# Autodesk Inventor assembly: feildAssembly
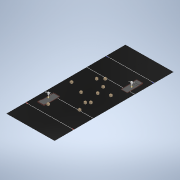
[picture p0: Inventor's stored thumbnail of the model, 180x180]
Saved by Autodesk Inventor 2020.3 (Build 243373000, 373)
## iProperties
Created: 2021-02-25
Part Number: feildAssembly
Document SubType Name: Assembly
Designer: con_c_000
Author: con_c_000
## iProperties of the stored document BlueAllianceTape-ver1-1111-2021.ipt
Created: 2019-10-14
Part Number: BlueAllianceTape-ver1-1111-2021
Material: Generic
Document SubType Name: Modeling
Designer: Phillips Lenovo
Density: 1 g/cm^3
Appearance: Default
Sending System: Autodesk Inventor 2021
Author: Phillips Lenovo
Revision Number: ANY
## iProperties of the stored document RedAllianceTape-ver1-1111-2021.ipt
Created: 2019-10-14
Part Number: RedAllianceTape-ver1-1111-2021
Material: Polyethylene, High Density
Document SubType Name: Modeling
Designer: Phillips Lenovo
Density: 0.952 g/cm^3
Appearance: Default
Sending System: Autodesk Inventor 2021
Author: Phillips Lenovo
Revision Number: ANY
## iProperties of the stored document FieldFloor-ver1-1111-2021.ipt
Created: 2019-10-14
Part Number: FieldFloor-ver1-1111-2021
Material: Polystyrene, High Impact
Document SubType Name: Modeling
Designer: Phillips Lenovo
Density: 1.022 g/cm^3
Appearance: Default
Sending System: Autodesk Inventor 2021
Author: Phillips Lenovo
Revision Number: ANY
## iProperties of the stored document Tape.ipt
Created: 2019-10-14
Part Number: Tape
Material: Generic
Document SubType Name: Modeling
Designer: Phillips Lenovo
Density: 1 g/cm^3
Appearance: Default
Sending System: Autodesk Inventor 2021
Author: Phillips Lenovo
Revision Number: ANY
## iProperties of the stored document ShipDesign-ver3-1111-2021.ipt
Created: 2021-02-04
Part Number: ShipDesign-ver3-1111-2021
Material: Wood (Oak)
Document SubType Name: Modeling
Designer: CMurray
Density: 0.76 g/cm^3
Appearance: Default
Sending System: Autodesk Inventor 2021
Author: CMurray
## iProperties of the stored document FullField-ver1-1111-2021.iam
Created: 2021-02-23
Part Number: FullField-ver2-1111-2021
Document SubType Name: Assembly
Designer: CMurray
Sending System: Autodesk Inventor 2021
Author: CMurray
## Documents named in this file (17)
- C:\Users\con_c_000\Documents\Inventor\Content Center Files\FIRST ROBOT\feildAssembly.iam
- **C:\Users\con_c_000\Documents\Inventor\Content Center Files\FIRST ROBOT\feildAssembly.iam*LocalDocs*xAaaaqtaaAaaaaaaaAaaaqz34Da*FullField-ver1-1111-2021.iam
- **C:\Users\con_c_000\Documents\Inventor\Content Center Files\FIRST ROBOT\feildAssembly.iam*LocalDocs*xAaaaqraaAaaaaaaaAaaaq1tgDa*ShipDesign-ver3-1111-2021.ipt
- C:\Users\con_c_000\Documents\Inventor\Content Center Files\FIRST ROBOT\cargoPrototype.ipt
- C:\Users\con_c_000\Documents\GitHub\RoboticsCad1111\PHRC CADD\2021 design challenge\capistan.iam
- C:\Users\con_c_000\Documents\GitHub\RoboticsCad1111\PHRC CADD\2021 design challenge\2021 Game Design Challenge\Full Field\Final Assembly\FullField-ver1-1111-2021.iam
- C:\Users\con_c_000\Documents\GitHub\RoboticsCad1111\PHRC CADD\2021 design challenge\2021 Game Design Challenge\Full Field\Parts\Tape\BlueAllianceTape-ver1-1111-2021.ipt
- C:\Users\con_c_000\Documents\GitHub\RoboticsCad1111\PHRC CADD\2021 design challenge\2021 Game Design Challenge\Full Field\Parts\FieldFloor-ver1-1111-2021.ipt
- C:\Users\con_c_000\Documents\GitHub\RoboticsCad1111\PHRC CADD\2021 design challenge\2021 Game Design Challenge\Full Field\Parts\Tape\RedAllianceTape-ver1-1111-2021.ipt
- C:\Users\con_c_000\Documents\GitHub\RoboticsCad1111\PHRC CADD\2021 design challenge\2021 Game Design Challenge\Full Field\Parts\Tape\Tape.ipt
- C:\Users\con_c_000\Documents\GitHub\RoboticsCad1111\PHRC CADD\2021 design challenge\2021 Game Design Challenge\Main Ship\ShipDesign-ver3-1111-2021.ipt
- **C:\Users\con_c_000\Documents\Inventor\Content Center Files\FIRST ROBOT\Assembly2.iam*LocalDocs*xAaaaamaaAaaaaaaaAaaaqlg43d*BlueAllianceTape-ver1-1111-2021.ipt
- **C:\Users\con_c_000\Documents\Inventor\Content Center Files\FIRST ROBOT\Assembly2.iam*LocalDocs*xAaaaamaaAaaaaaaaAaaaq0bkSa*RedAllianceTape-ver1-1111-2021.ipt
- **C:\Users\con_c_000\Documents\Inventor\Content Center Files\FIRST ROBOT\Assembly2.iam*LocalDocs*xAaaaqldaAaaaaaaaAaaaqmdqKf*FieldFloor-ver1-1111-2021.ipt
- **C:\Users\con_c_000\Documents\Inventor\Content Center Files\FIRST ROBOT\Assembly2.iam*LocalDocs*xAaaaqkcaAaaaaaaaAaaaq5yoYe*Tape.ipt
- **C:\Users\con_c_000\Documents\Inventor\Content Center Files\FIRST ROBOT\Assembly2.iam*LocalDocs*xAaaaqraaAaaaaaaaAaaaq1tgDa*ShipDesign-ver3-1111-2021.ipt
- **C:\Users\con_c_000\Documents\Inventor\Content Center Files\FIRST ROBOT\Assembly2.iam*LocalDocs*xAaaaqtaaAaaaaaaaAaaaqz34Da*FullField-ver1-1111-2021.iam
## Components (16 placed, 4 different names)
1. FullField-ver1-1111-2021:1 [sub-assembly] — Mate:1, Mate:4
2. ShipDesign-ver3-1111-2021:1 — Mate:4
3. ShipDesign-ver3-1111-2021:2 — Mate:1
4. cargoPrototype:1
5. cargoPrototype:2
6. cargoPrototype:3
7. cargoPrototype:4
8. cargoPrototype:5
9. cargoPrototype:6
10. cargoPrototype:7
11. cargoPrototype:8
12. cargoPrototype:9
13. cargoPrototype:10
14. cargoPrototype:11
15. capistan:1 [sub-assembly]
16. capistan:2 [sub-assembly]
## Relationships (2: Mate 2)
- Mate:1: FullField-ver1-1111-2021:1 ↔ ShipDesign-ver3-1111-2021:2
- Mate:4: FullField-ver1-1111-2021:1 ↔ ShipDesign-ver3-1111-2021:1
